# Autodesk Inventor assembly: Red Pump Assembly
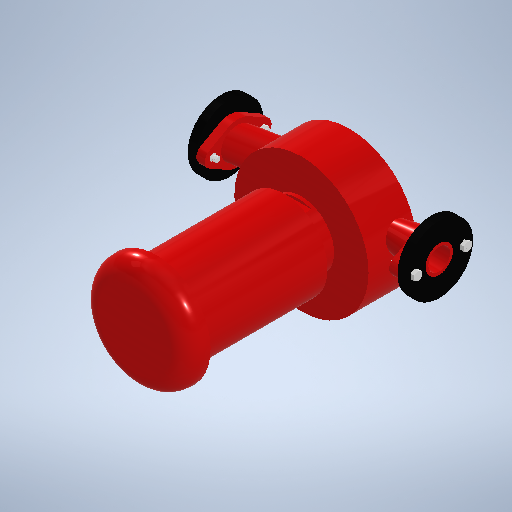
[picture p0: Inventor's stored thumbnail of the model, 512x512]
Saved by Autodesk Inventor 2027 (Build 310192000, 192)
## iProperties
Created: 2026-09-05
Part Number: Red Pump Assembly
Document SubType Name: Assembly
Designer: IG2
Author: IG2
## Documents named in this file (5)
- C:\Users\ig2\Desktop\Inventor stuff on your own\Red Pump Assembly.iam
- C:\Users\ig2\Desktop\SMR Thermal\thermal-loop\resources\v0.1.2\CAD\Inventor\aa FINAL MODEL with proportional valve\Red Pump.ipt
- C:\Users\ig2\Desktop\Inventor stuff on your own\Stainless Steel Left-Hand-Thread Hex Nut.ipt
- C:\Users\ig2\Desktop\Inventor stuff on your own\Medium-Strength Grade 5 Steel Hex Head Screw.ipt
- C:\Users\ig2\Desktop\Inventor stuff on your own\Red Pump Flange.ipt
## Components (11 placed, 4 different names)
1. Red Pump:1 — Rotational:1, Rigid:1, Rotational:5, Rotational:10, Rotational:11, Rotational:12
2. Stainless Steel Left-Hand-Thread Hex Nut:1 — Rotational:12
3. Stainless Steel Left-Hand-Thread Hex Nut:2 — Rotational:10
4. Stainless Steel Left-Hand-Thread Hex Nut:3 — Rotational:11
5. Stainless Steel Left-Hand-Thread Hex Nut:4 — Rigid:1
6. Medium-Strength Grade 5 Steel Hex Head Screw:1 — Rotational:9
7. Medium-Strength Grade 5 Steel Hex Head Screw:2 — Rotational:7
8. Medium-Strength Grade 5 Steel Hex Head Screw:3 — Rotational:8
9. Medium-Strength Grade 5 Steel Hex Head Screw:4 — Rotational:4
10. Red Pump Flange:1 — Rotational:5, Rotational:7, Rotational:8
11. Red Pump Flange:2 — Rotational:1, Rotational:4, Rotational:9
## Relationships (10: RevoluteJoint 9, WeldJoint 1)
- Rotational:1 [RevoluteJoint]: Red Pump:1 ↔ Red Pump Flange:2
- Rotational:4 [RevoluteJoint]: Medium-Strength Grade 5 Steel Hex Head Screw:4 ↔ Red Pump Flange:2
- Rigid:1 [WeldJoint]: Red Pump:1 ↔ Stainless Steel Left-Hand-Thread Hex Nut:4
- Rotational:5 [RevoluteJoint]: Red Pump:1 ↔ Red Pump Flange:1
- Rotational:7 [RevoluteJoint]: Medium-Strength Grade 5 Steel Hex Head Screw:2 ↔ Red Pump Flange:1
- Rotational:8 [RevoluteJoint]: Medium-Strength Grade 5 Steel Hex Head Screw:3 ↔ Red Pump Flange:1
- Rotational:9 [RevoluteJoint]: Medium-Strength Grade 5 Steel Hex Head Screw:1 ↔ Red Pump Flange:2
- Rotational:10 [RevoluteJoint]: Red Pump:1 ↔ Stainless Steel Left-Hand-Thread Hex Nut:2
- Rotational:11 [RevoluteJoint] (-5.08 mm): Red Pump:1 ↔ Stainless Steel Left-Hand-Thread Hex Nut:3
- Rotational:12 [RevoluteJoint]: Red Pump:1 ↔ Stainless Steel Left-Hand-Thread Hex Nut:1
